# Autodesk Inventor assembly: ASY MSC 203 RIGHT BOARD
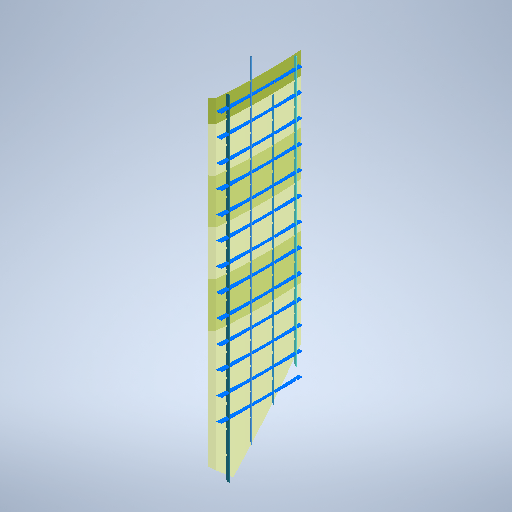
[picture p0: Inventor's stored thumbnail of the model, 512x512]
Saved by Autodesk Inventor 2025 (Build 290162010, 162A)
## iProperties
Created: 2024-07-22
Part Number: ASY MSC 203 RIGHT BOARD
Document SubType Name: Assembly
Designer: pokla
Author: pokla
## Documents named in this file (10)
- C:\Users\user\YandexDisk\домашниий пк\Inventor\Manturovo\Manturovo_Se-clar\ASY MSC 203 RIGHT BOARD.iam
- C:\Users\user\YandexDisk\домашниий пк\Inventor\Manturovo\Manturovo_Se-clar\MSC 052 rib board.ipt
- C:\Users\user\YandexDisk\домашниий пк\Inventor\Manturovo\Manturovo_Se-clar\MSC 024 sheet board main.ipt
- C:\Users\user\YandexDisk\домашниий пк\Inventor\Manturovo\Manturovo_Se-clar\MSC 023 sheet board.ipt
- C:\Users\user\YandexDisk\домашниий пк\Inventor\Manturovo\Manturovo_Se-clar\MSC 063 stringer board #.ipt
- C:\Users\user\YandexDisk\домашниий пк\Inventor\Manturovo\Manturovo_Se-clar\MSC 064 stringer board ##.ipt
- C:\Users\user\YandexDisk\домашниий пк\Inventor\Manturovo\Manturovo_Se-clar\MSC 065 stringer board ###.ipt
- C:\Users\user\YandexDisk\домашниий пк\Inventor\Manturovo\Manturovo_Se-clar\MSC 066 stringer board ####.ipt
- C:\Users\user\YandexDisk\домашниий пк\Inventor\Manturovo\Manturovo_Se-clar\MSC 026 sheet board withers 2.ipt
- C:\Users\user\YandexDisk\домашниий пк\Inventor\Manturovo\Manturovo_Se-clar\MSC 028 sheet board face 2.ipt
## Components (39 placed, 14 different names)
1. MSC 052 rib board.ipt:1 — Rigid:16
2. MSC 024 sheet board main.ipt:6
3. MSC 024 sheet board main.ipt:7
4. MSC 024 sheet board main.ipt:8
5. MSC 024 sheet board main.ipt:9
6. MSC 024 sheet board main.ipt:10 — Flush:2, Flush:3
7. MSC 023 sheet board.ipt:2
8. MSC 065 stringer board ###.ipt:1
9. MSC 066 stringer board ####.ipt:1
10. MSC 026 sheet board withers 2.ipt:1
11. MSC 028 sheet board face 2.ipt:1
12. MSC 052 rib board.ipt:4 — Rigid:16, Flush:1, Flush:2, Flush:3, Rigid:31
13. MSC 063 stringer board #.ipt:4 — Rigid:19
14. MSC 064 stringer board ##.ipt:4 — Rigid:22
15. MSC 065 stringer board ###.ipt:4 — Rigid:25
16. MSC 066 stringer board ####.ipt:4 — Rigid:28
17. МОО 053 стрингер борт 3:3 — Rigid:19, Rigid:20
18. МОО 053 стрингер борт 3:5 — Rigid:20, Rigid:21
19. МОО 053 стрингер борт 3:6 — Rigid:21
20. МОО 054 стрингер борт 4:3 — Rigid:22, Rigid:23
21. МОО 054 стрингер борт 4:5 — Rigid:23, Rigid:24
22. МОО 054 стрингер борт 4:6 — Rigid:24
23. МОО 055 стрингер борт 5:3 — Rigid:25, Rigid:26
24. МОО 055 стрингер борт 5:5 — Rigid:26, Rigid:27
25. МОО 055 стрингер борт 5:6 — Rigid:27
26. МОО 056 стрингер борт 6:3 — Rigid:28, Rigid:29
27. МОО 056 стрингер борт 6:5 — Rigid:29, Rigid:30
28. МОО 056 стрингер борт 6:6 — Rigid:30
29. MSC 052 rib board:3 — Rigid:31, Rigid:32
30. MSC 052 rib board:5 — Rigid:32, Rigid:33
31. MSC 052 rib board:6 — Rigid:33, Rigid:34
32. MSC 052 rib board:7 — Rigid:34, Rigid:38
33. MSC 052 rib board:8 — Rigid:38
34. MSC 052 rib board:9
35. MSC 052 rib board:10
36. MSC 052 rib board:11 — Rigid:41
37. MSC 052 rib board:12 — Rigid:41
38. MSC 052 rib board:13
39. MSC 052 rib board:14
## Relationships (39: WeldJoint 36, Flush 3)
- [WeldJoint]: MSC 024 sheet board main.ipt:6 ↔ MSC 024 sheet board main.ipt:7
- [WeldJoint]: MSC 024 sheet board main.ipt:7 ↔ MSC 024 sheet board main.ipt:8
- [WeldJoint]: MSC 024 sheet board main.ipt:8 ↔ MSC 024 sheet board main.ipt:9
- [WeldJoint]: MSC 024 sheet board main.ipt:9 ↔ MSC 024 sheet board main.ipt:10
- [WeldJoint]: MSC 024 sheet board main.ipt:10 ↔ MSC 023 sheet board.ipt:2
- [WeldJoint]: MSC 026 sheet board withers 2.ipt:1 ↔ MSC 028 sheet board face 2.ipt:1
- [WeldJoint]: MSC 024 sheet board main.ipt:6 ↔ MSC 026 sheet board withers 2.ipt:1
- [WeldJoint]: MSC 065 stringer board ###.ipt:1 ↔ MSC 065 stringer board ###.ipt:4
- [WeldJoint]: MSC 066 stringer board ####.ipt:1 ↔ MSC 066 stringer board ####.ipt:4
- [WeldJoint] (2 mm): MSC 052 rib board.ipt:1 ↔ MSC 063 stringer board #.ipt:4
- [WeldJoint] (2 mm): MSC 052 rib board.ipt:1 ↔ MSC 066 stringer board ####.ipt:1
- [WeldJoint] (2 mm): MSC 052 rib board.ipt:1 ↔ MSC 065 stringer board ###.ipt:1
- Rigid:16 [WeldJoint] (-500 mm): MSC 052 rib board.ipt:1 ↔ MSC 052 rib board.ipt:4
- Flush:1: MSC 052 rib board.ipt:4
- Flush:2 (250 mm): MSC 024 sheet board main.ipt:10 ↔ MSC 052 rib board.ipt:4
- Flush:3: MSC 024 sheet board main.ipt:10 ↔ MSC 052 rib board.ipt:4
- Rigid:19 [WeldJoint]: MSC 063 stringer board #.ipt:4 ↔ МОО 053 стрингер борт 3:3
- Rigid:20 [WeldJoint]: МОО 053 стрингер борт 3:3 ↔ МОО 053 стрингер борт 3:5
- Rigid:21 [WeldJoint]: МОО 053 стрингер борт 3:5 ↔ МОО 053 стрингер борт 3:6
- Rigid:22 [WeldJoint]: MSC 064 stringer board ##.ipt:4 ↔ МОО 054 стрингер борт 4:3
- Rigid:23 [WeldJoint]: МОО 054 стрингер борт 4:3 ↔ МОО 054 стрингер борт 4:5
- Rigid:24 [WeldJoint]: МОО 054 стрингер борт 4:5 ↔ МОО 054 стрингер борт 4:6
- Rigid:25 [WeldJoint]: MSC 065 stringer board ###.ipt:4 ↔ МОО 055 стрингер борт 5:3
- Rigid:26 [WeldJoint]: МОО 055 стрингер борт 5:3 ↔ МОО 055 стрингер борт 5:5
- Rigid:27 [WeldJoint]: МОО 055 стрингер борт 5:5 ↔ МОО 055 стрингер борт 5:6
- Rigid:28 [WeldJoint]: MSC 066 stringer board ####.ipt:4 ↔ МОО 056 стрингер борт 6:3
- Rigid:29 [WeldJoint]: МОО 056 стрингер борт 6:3 ↔ МОО 056 стрингер борт 6:5
- Rigid:30 [WeldJoint]: МОО 056 стрингер борт 6:5 ↔ МОО 056 стрингер борт 6:6
- Rigid:31 [WeldJoint] (-500 mm): MSC 052 rib board.ipt:4 ↔ MSC 052 rib board:3
- Rigid:32 [WeldJoint] (-500 mm): MSC 052 rib board:3 ↔ MSC 052 rib board:5
- Rigid:33 [WeldJoint] (-500 mm): MSC 052 rib board:5 ↔ MSC 052 rib board:6
- Rigid:34 [WeldJoint] (-500 mm): MSC 052 rib board:6 ↔ MSC 052 rib board:7
- [WeldJoint] (-500 mm): MSC 052 rib board:8 ↔ MSC 052 rib board:9
- [WeldJoint] (-500 mm): MSC 052 rib board:9 ↔ MSC 052 rib board:10
- [WeldJoint] (-500 mm): MSC 052 rib board:10 ↔ MSC 052 rib board:11
- Rigid:38 [WeldJoint] (-500 mm): MSC 052 rib board:7 ↔ MSC 052 rib board:8
- [WeldJoint] (-500 mm): MSC 052 rib board:12 ↔ MSC 052 rib board:13
- [WeldJoint] (-500 mm): MSC 052 rib board:13 ↔ MSC 052 rib board:14
- Rigid:41 [WeldJoint] (-500 mm): MSC 052 rib board:11 ↔ MSC 052 rib board:12
## Named parameters: d230_d194 = 0 mm, d231_d195 = 0 mm, d232_d160 = 0 mm, d233_d161 = 0 mm, d39_d36 = -500 mm, d40_d37 = -500 mm, d41_d38 = -500 mm, d43_d40_d37 = -500 mm, d44_d41_d38 = -500 mm
